# Autodesk Inventor assembly: 4x2020_in
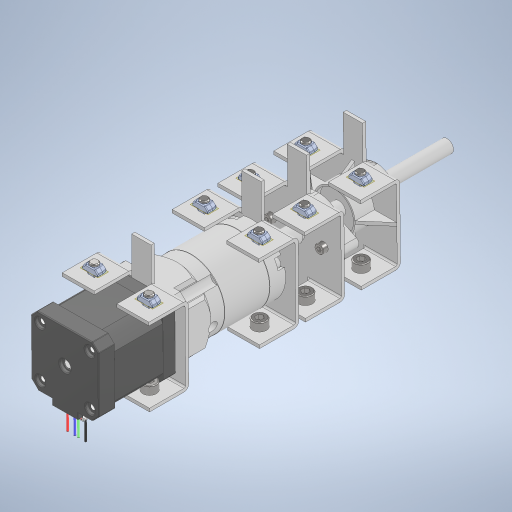
[picture p0: Inventor's stored thumbnail of the model, 512x512]
Saved by Autodesk Inventor 2024 (Build 280153000, 153)
## iProperties
Created: 2025-12-16
Part Number: 4x2020_in
Document SubType Name: Assembly
Designer: schar
Author: schar
## Documents named in this file (11)
- C:\Users\schar\Desktop\projectBlueprint\AMSTS\hardware\4x2020_in.iam
- C:\Users\schar\Desktop\projectBlueprint\AMSTS\hardware\4x2020_universal.ipt
- C:\Users\schar\Desktop\projectBlueprint\AMSTS\hardware\17HE19-2004S.ipt
- C:\Users\schar\Desktop\projectBlueprint\AMSTS\hardware\4x2020_universal_planetary.ipt
- C:\Users\schar\Desktop\projectBlueprint\AMSTS\hardware\EG17-G20.iam
- C:\Users\schar\Desktop\projectBlueprint\AMSTS\hardware\4x2020_axis.ipt
- C:\Users\schar\Desktop\projectBlueprint\AMSTS\hardware\4x2020_encoder.iam
- C:\Users\schar\Desktop\projectBlueprint\AMSTS\hardware\4x2020_axis_end_bearings.ipt
- C:\Users\schar\Desktop\projectBlueprint\AMSTS\hardware\628_bearing.ipt
- C:\Users\schar\Desktop\projectBlueprint\AMSTS\hardware\tnut_m5_2020.ipt
- C:\Users\schar\Documents\Inventor\Content Center Files\R2024\en-US\ISO 4762(1)\DIN EN ISO 4762 - M5 x 8.ipt
## Components (41 placed, 10 different names)
1. 4x2020_universal:1 — Mate:1, Mate:2, Mate:3, Mate:4, Mate:5, Mate:6, Rotational:1, Rotational:4, Symmetry:1, Rotational:9, Rotational:13, Mate:20, Mate:21, Mate:34, Mate:35, Mate:36, Mate:37, Mate:38, Mate:39
2. 17HE19-2004S:1 — Mate:1, Mate:2, Mate:3
3. 4x2020_universal_planetary:1 — Mate:7, Mate:8, Mate:9, Rotational:2, Rotational:5, Symmetry:1, Rotational:10, Rotational:14, Mate:22, Mate:23, Mate:32, Mate:33, Mate:40, Mate:41, Mate:42, Mate:43
4. EG17-G20:1 [sub-assembly] — Mate:4, Mate:5, Mate:6, Mate:7, Mate:8, Mate:9, Mate:10, Mate:11
5. 4x2020_axis:1 — Mate:10, Mate:11, Mate:12, Mate:13, Mate:18
6. 4x2020_encoder:1 [sub-assembly] — Mate:12, Mate:13, Mate:19, Rotational:6, Rotational:8, Rotational:11, Rotational:15, Mate:24, Mate:25, Mate:30, Mate:31, Mate:44, Mate:45, Mate:46, Mate:47
7. 4x2020_axis_end_bearings:1 — Mate:14, Mate:15, Mate:16, Mate:17, Mate:18, Mate:19, Rotational:3, Rotational:7, Rotational:12, Rotational:16, Mate:26, Mate:27, Mate:28, Mate:29, Mate:48, Mate:49, Mate:50, Mate:51
8. 628_bearing:1 — Mate:16, Mate:17
9. 628_bearing:2 — Mate:14, Mate:15
10. tnut_m5_2020:1 — Rotational:1
11. tnut_m5_2020:2 — Rotational:4
12. tnut_m5_2020:3 — Rotational:5
13. tnut_m5_2020:4 — Rotational:6
14. tnut_m5_2020:5 — Rotational:3
15. tnut_m5_2020:6 — Rotational:8
16. tnut_m5_2020:7 — Rotational:2
17. tnut_m5_2020:8 — Rotational:7
18. tnut_m5_2020:9 — Rotational:9
19. tnut_m5_2020:10 — Rotational:10
20. tnut_m5_2020:11 — Rotational:11
21. tnut_m5_2020:12 — Rotational:12
22. tnut_m5_2020:13 — Rotational:13
23. tnut_m5_2020:14 — Rotational:14
24. tnut_m5_2020:15 — Rotational:15
25. tnut_m5_2020:16 — Rotational:16
26. DIN EN ISO 4762 M5 x 8:1 — Mate:20, Mate:21
27. DIN EN ISO 4762 M5 x 8:2 — Mate:22, Mate:23
28. DIN EN ISO 4762 M5 x 8:3 — Mate:24, Mate:25
29. DIN EN ISO 4762 M5 x 8:4 — Mate:26, Mate:27
30. DIN EN ISO 4762 M5 x 8:5 — Mate:34, Mate:35
31. DIN EN ISO 4762 M5 x 8:6 — Mate:32, Mate:33
32. DIN EN ISO 4762 M5 x 8:7 — Mate:30, Mate:31
33. DIN EN ISO 4762 M5 x 8:8 — Mate:28, Mate:29
34. DIN EN ISO 4762 M5 x 8:9 — Mate:36, Mate:37
35. DIN EN ISO 4762 M5 x 8:10 — Mate:38, Mate:39
36. DIN EN ISO 4762 M5 x 8:11 — Mate:40, Mate:41
37. DIN EN ISO 4762 M5 x 8:12 — Mate:42, Mate:43
38. DIN EN ISO 4762 M5 x 8:13 — Mate:44, Mate:45
39. DIN EN ISO 4762 M5 x 8:14 — Mate:46, Mate:47
40. DIN EN ISO 4762 M5 x 8:15 — Mate:48, Mate:49
41. DIN EN ISO 4762 M5 x 8:16 — Mate:50, Mate:51
## Relationships (68: Mate 51, RevoluteJoint 16, Symmetry 1)
- Mate:1: 4x2020_universal:1 ↔ 17HE19-2004S:1
- Mate:2: 4x2020_universal:1 ↔ 17HE19-2004S:1
- Mate:3: 4x2020_universal:1 ↔ 17HE19-2004S:1
- Mate:4: 4x2020_universal:1 ↔ EG17-G20:1
- Mate:5: 4x2020_universal:1 ↔ EG17-G20:1
- Mate:6: 4x2020_universal:1 ↔ EG17-G20:1
- Mate:7: 4x2020_universal_planetary:1 ↔ EG17-G20:1
- Mate:8: 4x2020_universal_planetary:1 ↔ EG17-G20:1
- Mate:9: 4x2020_universal_planetary:1 ↔ EG17-G20:1
- Mate:10: EG17-G20:1 ↔ 4x2020_axis:1
- Mate:11: EG17-G20:1 ↔ 4x2020_axis:1
- Mate:12 (2 mm): 4x2020_axis:1 ↔ 4x2020_encoder:1
- Mate:13: 4x2020_axis:1 ↔ 4x2020_encoder:1
- Mate:14: 4x2020_axis_end_bearings:1 ↔ 628_bearing:2
- Mate:15: 4x2020_axis_end_bearings:1 ↔ 628_bearing:2
- Mate:16: 4x2020_axis_end_bearings:1 ↔ 628_bearing:1
- Mate:17: 4x2020_axis_end_bearings:1 ↔ 628_bearing:1
- Mate:18: 4x2020_axis:1 ↔ 4x2020_axis_end_bearings:1
- Mate:19: 4x2020_encoder:1 ↔ 4x2020_axis_end_bearings:1
- Rotational:1 [RevoluteJoint] (-0.159 mm): 4x2020_universal:1 ↔ tnut_m5_2020:1
- Rotational:2 [RevoluteJoint] (-0.159 mm): 4x2020_universal_planetary:1 ↔ tnut_m5_2020:7
- Rotational:3 [RevoluteJoint] (-0.159 mm): 4x2020_axis_end_bearings:1 ↔ tnut_m5_2020:5
- Rotational:4 [RevoluteJoint] (-0.159 mm): 4x2020_universal:1 ↔ tnut_m5_2020:2
- Rotational:5 [RevoluteJoint] (-0.159 mm): 4x2020_universal_planetary:1 ↔ tnut_m5_2020:3
- Rotational:6 [RevoluteJoint] (-0.159 mm): 4x2020_encoder:1 ↔ tnut_m5_2020:4
- Rotational:7 [RevoluteJoint] (-0.159 mm): 4x2020_axis_end_bearings:1 ↔ tnut_m5_2020:8
- Symmetry:1: 4x2020_universal:1 ↔ 4x2020_universal_planetary:1
- Rotational:8 [RevoluteJoint] (-0.159 mm): 4x2020_encoder:1 ↔ tnut_m5_2020:6
- Rotational:9 [RevoluteJoint] (-0.159 mm): 4x2020_universal:1 ↔ tnut_m5_2020:9
- Rotational:10 [RevoluteJoint] (-0.159 mm): 4x2020_universal_planetary:1 ↔ tnut_m5_2020:10
- Rotational:11 [RevoluteJoint] (-0.159 mm): 4x2020_encoder:1 ↔ tnut_m5_2020:11
- Rotational:12 [RevoluteJoint] (-0.159 mm): 4x2020_axis_end_bearings:1 ↔ tnut_m5_2020:12
- Rotational:13 [RevoluteJoint] (-0.159 mm): 4x2020_universal:1 ↔ tnut_m5_2020:13
- Rotational:14 [RevoluteJoint] (-0.159 mm): 4x2020_universal_planetary:1 ↔ tnut_m5_2020:14
- Rotational:15 [RevoluteJoint] (-0.159 mm): 4x2020_encoder:1 ↔ tnut_m5_2020:15
- Rotational:16 [RevoluteJoint] (-0.159 mm): 4x2020_axis_end_bearings:1 ↔ tnut_m5_2020:16
- Mate:20: 4x2020_universal:1 ↔ DIN EN ISO 4762 M5 x 8:1
- Mate:21: 4x2020_universal:1 ↔ DIN EN ISO 4762 M5 x 8:1
- Mate:22: 4x2020_universal_planetary:1 ↔ DIN EN ISO 4762 M5 x 8:2
- Mate:23: 4x2020_universal_planetary:1 ↔ DIN EN ISO 4762 M5 x 8:2
- Mate:24: 4x2020_encoder:1 ↔ DIN EN ISO 4762 M5 x 8:3
- Mate:25: 4x2020_encoder:1 ↔ DIN EN ISO 4762 M5 x 8:3
- Mate:26: 4x2020_axis_end_bearings:1 ↔ DIN EN ISO 4762 M5 x 8:4
- Mate:27: 4x2020_axis_end_bearings:1 ↔ DIN EN ISO 4762 M5 x 8:4
- Mate:28: 4x2020_axis_end_bearings:1 ↔ DIN EN ISO 4762 M5 x 8:8
- Mate:29: 4x2020_axis_end_bearings:1 ↔ DIN EN ISO 4762 M5 x 8:8
- Mate:30: 4x2020_encoder:1 ↔ DIN EN ISO 4762 M5 x 8:7
- Mate:31: 4x2020_encoder:1 ↔ DIN EN ISO 4762 M5 x 8:7
- Mate:32: 4x2020_universal_planetary:1 ↔ DIN EN ISO 4762 M5 x 8:6
- Mate:33: 4x2020_universal_planetary:1 ↔ DIN EN ISO 4762 M5 x 8:6
- Mate:34: 4x2020_universal:1 ↔ DIN EN ISO 4762 M5 x 8:5
- Mate:35: 4x2020_universal:1 ↔ DIN EN ISO 4762 M5 x 8:5
- Mate:36: 4x2020_universal:1 ↔ DIN EN ISO 4762 M5 x 8:9
- Mate:37: 4x2020_universal:1 ↔ DIN EN ISO 4762 M5 x 8:9
- Mate:38: 4x2020_universal:1 ↔ DIN EN ISO 4762 M5 x 8:10
- Mate:39: 4x2020_universal:1 ↔ DIN EN ISO 4762 M5 x 8:10
- Mate:40: 4x2020_universal_planetary:1 ↔ DIN EN ISO 4762 M5 x 8:11
- Mate:41: 4x2020_universal_planetary:1 ↔ DIN EN ISO 4762 M5 x 8:11
- Mate:42: 4x2020_universal_planetary:1 ↔ DIN EN ISO 4762 M5 x 8:12
- Mate:43: 4x2020_universal_planetary:1 ↔ DIN EN ISO 4762 M5 x 8:12
- Mate:44: 4x2020_encoder:1 ↔ DIN EN ISO 4762 M5 x 8:13
- Mate:45: 4x2020_encoder:1 ↔ DIN EN ISO 4762 M5 x 8:13
- Mate:46: 4x2020_encoder:1 ↔ DIN EN ISO 4762 M5 x 8:14
- Mate:47: 4x2020_encoder:1 ↔ DIN EN ISO 4762 M5 x 8:14
- Mate:48: 4x2020_axis_end_bearings:1 ↔ DIN EN ISO 4762 M5 x 8:15
- Mate:49: 4x2020_axis_end_bearings:1 ↔ DIN EN ISO 4762 M5 x 8:15
- Mate:50: 4x2020_axis_end_bearings:1 ↔ DIN EN ISO 4762 M5 x 8:16
- Mate:51: 4x2020_axis_end_bearings:1 ↔ DIN EN ISO 4762 M5 x 8:16
